# Autodesk Inventor assembly: Intake Full Assembly
(part 2 of 2)
- Mate:583: Intake Roller Plate:1 ↔ COTS_92949A265_1-2in long Stainless Steel Button Head Screw:9
- Mate:584: Intake Roller Plate:1 ↔ COTS_92949A265_1-2in long Stainless Steel Button Head Screw:21
- Mate:585: Intake Roller Plate:1 ↔ COTS_92949A265_1-2in long Stainless Steel Button Head Screw:19
- Mate:586: Intake Roller Plate:1 ↔ COTS_92949A265_1-2in long Stainless Steel Button Head Screw:6
- Mate:587: Intake Roller Plate:1 ↔ COTS_92949A265_1-2in long Stainless Steel Button Head Screw:20
- Mate:588: Intake Roller Plate:1 ↔ COTS_92949A265_1-2in long Stainless Steel Button Head Screw:8
- Mate:589: INTK_001_PulleyCover:1 ↔ COTS_92949A265_1-2in long Stainless Steel Button Head Screw:14
- Mate:590: INTK_001_PulleyCover:1 ↔ COTS_92949A265_1-2in long Stainless Steel Button Head Screw:15
- Mate:591: INTK_001_PulleyCover:1 ↔ COTS_92949A265_1-2in long Stainless Steel Button Head Screw:24
- Mate:592: INTK_001_PulleyCover:1 ↔ COTS_92949A265_1-2in long Stainless Steel Button Head Screw:17
- Mate:593: INTK_001_PulleyCover:1 ↔ COTS_92949A265_1-2in long Stainless Steel Button Head Screw:18
- Mate:594: INTK_001_PulleyCover:1 ↔ COTS_92949A265_1-2in long Stainless Steel Button Head Screw:7
- Mate:595: INTK_001_PulleyCover:1 ↔ COTS_92949A265_1-2in long Stainless Steel Button Head Screw:16
- Mate:596: INTK_001_PulleyCover:2 ↔ COTS_92949A265_1-2in long Stainless Steel Button Head Screw:2
- Mate:597: INTK_001_PulleyCover:2 ↔ COTS_92949A265_1-2in long Stainless Steel Button Head Screw:5
- Mate:598: INTK_001_PulleyCover:2 ↔ COTS_92949A265_1-2in long Stainless Steel Button Head Screw:4
- Mate:599: INTK_001_PulleyCover:2 ↔ COTS_92949A265_1-2in long Stainless Steel Button Head Screw:1
- Mate:600: INTK_001_PulleyCover:2 ↔ COTS_92949A265_1-2in long Stainless Steel Button Head Screw:12
- Mate:601: INTK_001_PulleyCover:2 ↔ COTS_92949A265_1-2in long Stainless Steel Button Head Screw:13
- Mate:602: INTK_001_PulleyCover:2 ↔ COTS_92949A265_1-2in long Stainless Steel Button Head Screw:3
- Mate:603: INTK_001_PulleyCover:2 ↔ COTS_92949A265_1-2in long Stainless Steel Button Head Screw:13
- Mate:604: INTK_001_PulleyCover:2 ↔ COTS_92949A265_1-2in long Stainless Steel Button Head Screw:3
- Mate:605: INTK_001_PulleyCover:2 ↔ COTS_92949A265_1-2in long Stainless Steel Button Head Screw:1
- Mate:606: INTK_001_PulleyCover:2 ↔ COTS_92949A265_1-2in long Stainless Steel Button Head Screw:2
- Mate:607: INTK_001_PulleyCover:2 ↔ COTS_92949A265_1-2in long Stainless Steel Button Head Screw:5
- Mate:608: INTK_001_PulleyCover:2 ↔ COTS_92949A265_1-2in long Stainless Steel Button Head Screw:4
- Mate:609: INTK_001_PulleyCover:2 ↔ COTS_92949A265_1-2in long Stainless Steel Button Head Screw:12
- Mate:610: Intake Roller Plate:2 ↔ COTS_92949A265_1-2in long Stainless Steel Button Head Screw:26
- Mate:611: Intake Roller Plate:2 ↔ COTS_92949A265_1-2in long Stainless Steel Button Head Screw:11
- Mate:612: Intake Roller Plate:2 ↔ COTS_92949A265_1-2in long Stainless Steel Button Head Screw:25
- Mate:613: Intake Roller Plate:2 ↔ COTS_92949A265_1-2in long Stainless Steel Button Head Screw:27
- Mate:614: Intake Roller Plate:2 ↔ COTS_92949A265_1-2in long Stainless Steel Button Head Screw:23
- Mate:615: Intake Roller Plate:2 ↔ COTS_92949A265_1-2in long Stainless Steel Button Head Screw:22
- Mate:616: Intake Roller Plate:2 ↔ COTS_92949A265_1-2in long Stainless Steel Button Head Screw:26
- Mate:617: Intake Roller Plate:2 ↔ COTS_92949A265_1-2in long Stainless Steel Button Head Screw:22
- Mate:618: Intake Roller Plate:2 ↔ COTS_92949A265_1-2in long Stainless Steel Button Head Screw:23
- Mate:619: Intake Roller Plate:2 ↔ COTS_92949A265_1-2in long Stainless Steel Button Head Screw:27
- Mate:620: Intake Roller Plate:2 ↔ COTS_92949A265_1-2in long Stainless Steel Button Head Screw:25
- Mate:621: Intake Roller Plate:2 ↔ COTS_92949A265_1-2in long Stainless Steel Button Head Screw:11
